# Autodesk Inventor assembly: Caja_Reductora_
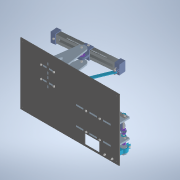
[picture p0: Inventor's stored thumbnail of the model, 180x180]
Saved by Autodesk Inventor 2022 (Build 260153000, 153)
## iProperties
Created: 2022-03-04
Part Number: Caja_Reductora_
Document SubType Name: Assembly
Designer: katha
Author: katha
## Documents named in this file (26)
- C:\Users\katha\OneDrive\Escritorio\Mini_Proyecto_Diseno\Diseno_18012\Modelo_MPD\Caja_Reductora_.iam
- C:\Users\katha\OneDrive\Escritorio\Mini_Proyecto_Diseno\Diseno_18012\Modelo_MPD\Carcasa_CajaR_Lateral1.ipt
- C:\Users\katha\OneDrive\Escritorio\Mini_Proyecto_Diseno\Diseno_18012\Modelo_MPD\Carcasa_Tope.ipt
- C:\Users\katha\OneDrive\Escritorio\Mini_Proyecto_Diseno\Diseno_18012\Modelo_MPD\M4_short.ipt
- C:\Users\katha\OneDrive\Escritorio\Mini_Proyecto_Diseno\Diseno_18012\Modelo_MPD\M4_tuerca.ipt
- C:\Users\katha\OneDrive\Escritorio\Mini_Proyecto_Diseno\Diseno_18012\Modelo_MPD\Rodamiento_Ejes.ipt
- C:\Users\katha\OneDrive\Escritorio\Mini_Proyecto_Diseno\Diseno_18012\Modelo_MPD\Eje_Entrada.ipt
- C:\Users\katha\OneDrive\Escritorio\Mini_Proyecto_Diseno\Diseno_18012\Modelo_MPD\Eje1.ipt
- C:\Users\katha\OneDrive\Escritorio\Mini_Proyecto_Diseno\Diseno_18012\Modelo_MPD\Eje2.ipt
- C:\Users\katha\OneDrive\Escritorio\Mini_Proyecto_Diseno\Diseno_18012\Modelo_MPD\Eje_Salida.ipt
- C:\Users\katha\OneDrive\Escritorio\Mini_Proyecto_Diseno\Diseno_18012\Modelo_MPD\Engranajes_60.ipt
- C:\Users\katha\OneDrive\Escritorio\Mini_Proyecto_Diseno\Diseno_18012\Modelo_MPD\Engranajes_15.ipt
- C:\Users\katha\OneDrive\Escritorio\Mini_Proyecto_Diseno\Diseno_18012\Modelo_MPD\Engranajes_12.ipt
- C:\Users\katha\OneDrive\Escritorio\Mini_Proyecto_Diseno\Diseno_18012\Modelo_MPD\Hombro_Ejes.ipt
- C:\Users\katha\OneDrive\Escritorio\Mini_Proyecto_Diseno\Diseno_18012\Modelo_MPD\pasador.ipt
- C:\Users\katha\OneDrive\Escritorio\Mini_Proyecto_Diseno\Diseno_18012\Modelo_MPD\Base_proyecto.ipt
- C:\Users\katha\OneDrive\Escritorio\Mini_Proyecto_Diseno\Diseno_18012\Modelo_MPD\Base.ipt
- C:\Users\katha\OneDrive\Escritorio\Mini_Proyecto_Diseno\Diseno_18012\Modelo_MPD\Base_Soporte.ipt
- C:\Users\katha\OneDrive\Escritorio\Mini_Proyecto_Diseno\Diseno_18012\Modelo_MPD\Carril.iam
- C:\Users\katha\OneDrive\Escritorio\Mini_Proyecto_Diseno\Diseno_18012\Modelo_MPD\Eslabon_TransPot.ipt
- C:\Users\katha\OneDrive\Escritorio\Mini_Proyecto_Diseno\Diseno_18012\Modelo_MPD\base_motor.ipt
- C:\Users\katha\OneDrive\Escritorio\Mini_Proyecto_Diseno\Diseno_18012\Modelo_MPD\motor.ipt
- C:\Users\katha\OneDrive\Escritorio\Mini_Proyecto_Diseno\Diseno_18012\Modelo_MPD\Acople_TransPot.ipt
- C:\Users\katha\OneDrive\Escritorio\Mini_Proyecto_Diseno\Diseno_18012\Modelo_MPD\Acople_Motor_.ipt
- C:\Users\katha\OneDrive\Escritorio\Mini_Proyecto_Diseno\Diseno_18012\Modelo_MPD\M4_long.ipt
- C:\Users\katha\OneDrive\Escritorio\Mini_Proyecto_Diseno\Diseno_18012\Modelo_MPD\rodamiento_carril.ipt
## Components (99 placed, 25 different names)
1. Carcasa_CajaR_Lateral1:1 — Flush:1, Flush:2, Mate:1, Mate:25, Mate:26, Mate:27, Mate:35, Mate:43, Mate:46, Mate:47, Flush:3, Mate:48, Mate:49, Mate:50, Mate:131, Mate:132, Flush:33
2. Carcasa_CajaR_Lateral1:2 — Flush:1, Flush:2, Mate:1, Mate:28, Mate:29, Mate:30, Mate:44, Mate:45, Mate:51, Mate:52, Mate:53, Mate:54, Flush:4, Mate:141, Mate:142, Mate:143, Mate:144
3. Carcasa_Tope:1 — Mate:25, Mate:26, Mate:27, Mate:33, Mate:34, Mate:36
4. Carcasa_Tope:2 — Mate:28, Mate:29, Mate:30, Mate:31, Mate:32, Mate:37, Mate:38
5. M4_short:1 — Mate:35, Mate:36, Mate:41
6. M4_short:2 — Mate:33, Mate:34, Mate:42
7. M4_short:3 — Mate:37, Mate:38, Mate:39
8. M4_short:4 — Mate:31, Mate:32, Mate:40
9. M4_tuerca:1 — Mate:39, Mate:45
10. M4_tuerca:2 — Mate:40, Mate:44
11. M4_tuerca:3 — Mate:42, Mate:43
12. M4_tuerca:4 — Mate:41, Mate:46
13. Rodamiento_Ejes:1 — Mate:48, Flush:8, Mate:59, Mate:60, Flush:12
14. Rodamiento_Ejes:2 — Mate:49, Flush:9, Mate:63, Mate:64, Flush:13
15. Rodamiento_Ejes:3 — Mate:51, Flush:4, Flush:5, Flush:6, Flush:7, Mate:57, Mate:58
16. Rodamiento_Ejes:4 — Mate:54, Flush:7, Mate:67, Mate:68, Flush:14
17. Rodamiento_Ejes:5 — Mate:53, Flush:6, Mate:65, Mate:66
18. Rodamiento_Ejes:6 — Mate:52, Flush:5, Mate:61, Mate:62
19. Rodamiento_Ejes:7 — Mate:50, Flush:10, Mate:69, Mate:70
20. Rodamiento_Ejes:8 — Mate:47, Flush:3, Flush:8, Flush:9, Flush:10, Mate:55, Mate:56, Flush:11
21. Eje_Entrada:1 — Mate:55, Mate:56, Mate:57, Mate:58, Flush:11, Mate:77, Mate:78, Flush:15, Mate:83, Mate:84, Mate:85, Mate:86, Mate:87, Mate:88, Mate:192, Mate:193, Mate:194
22. Eje1:1 — Mate:59, Mate:60, Mate:61, Mate:62, Flush:12, Mate:73, Mate:74, Mate:79, Mate:80, Flush:17, Mate:89, Mate:90, Mate:91, Mate:92, Mate:93, Mate:94, Mate:95, Mate:96, Mate:97, Mate:98, Mate:99, Mate:100
23. Eje2:1 — Mate:63, Mate:64, Mate:65, Mate:66, Flush:13, Mate:71, Mate:72, Mate:81, Mate:82, Flush:19, Mate:101, Mate:102, Mate:103, Mate:104, Mate:105, Mate:106, Mate:107, Mate:108, Mate:109, Mate:110, Mate:111, Mate:112
24. Eje_Salida:1 — Mate:67, Mate:68, Flush:14, Mate:69, Mate:70, Mate:75, Mate:76, Mate:113, Mate:114, Mate:115, Mate:116, Mate:117, Mate:118, Mate:183, Mate:184, Mate:185
25. Engranajes_60:1 — Mate:71, Mate:72, Flush:18
26. Engranajes_60:2 — Mate:73, Mate:74, Flush:16
27. Engranajes_60:3 — Mate:75, Mate:76, Flush:20
28. Engranajes_15:1 — Mate:77, Mate:78, Flush:15, Flush:16
29. Engranajes_15:2 — Mate:79, Mate:80, Flush:17, Flush:18
30. Engranajes_12:1 — Mate:81, Mate:82, Flush:19, Flush:20
31. Hombro_Ejes:1 — Mate:83, Mate:84, Mate:85, Mate:120, Flush:21
32. Hombro_Ejes:2 — Mate:86, Mate:87, Mate:88, Mate:119, Flush:22
33. Hombro_Ejes:3 — Mate:110, Mate:111, Mate:112, Mate:125, Flush:30
34. Hombro_Ejes:4 — Mate:95, Mate:96, Mate:97, Mate:123, Flush:24
35. Hombro_Ejes:5 — Mate:92, Mate:93, Mate:94, Mate:122, Flush:25
36. Hombro_Ejes:6 — Mate:107, Mate:108, Mate:109, Mate:126, Flush:32
37. Hombro_Ejes:7 — Mate:89, Mate:90, Mate:91, Mate:121, Flush:26
38. Hombro_Ejes:8 — Mate:98, Mate:99, Mate:100, Mate:124, Flush:23
39. Hombro_Ejes:9 — Mate:116, Mate:117, Mate:118, Mate:130, Flush:27
40. Hombro_Ejes:10 — Mate:101, Mate:102, Mate:103, Mate:128, Flush:29
41. Hombro_Ejes:11 — Mate:113, Mate:114, Mate:115, Mate:129, Flush:28
42. Hombro_Ejes:12 — Mate:104, Mate:105, Mate:106, Mate:127, Flush:31
43. pasador:1 — Mate:119, Flush:22
44. pasador:2 — Mate:120, Flush:21
45. pasador:3 — Mate:125, Flush:30
46. pasador:4 — Mate:126, Flush:32
47. pasador:5 — Mate:128, Flush:29
48. pasador:6 — Mate:130, Flush:27
49. pasador:7 — Mate:129, Flush:28
50. pasador:8 — Mate:127, Flush:31
51. pasador:9 — Mate:123, Flush:24
52. pasador:10 — Mate:121, Flush:26
53. pasador:11 — Mate:122, Flush:25
54. pasador:12 — Mate:124, Flush:23
55. Base_proyecto:1 — Mate:131, Mate:132, Flush:33, Mate:133, Mate:134, Mate:135, Mate:136, Mate:137, Mate:138, Mate:139, Mate:140, Mate:149, Mate:150, Mate:151, Mate:152, Flush:34, Flush:35, Mate:153, Mate:154, Flush:36, Mate:155, Mate:156, Mate:157, Mate:158, Mate:159, Mate:160, Mate:161, Mate:162, Mate:179, Mate:180, Mate:181, Mate:218, Mate:219
56. M4_short:5 — Mate:136, Mate:138, Mate:148
57. M4_short:6 — Mate:134, Mate:139, Mate:146
58. M4_short:7 — Mate:133, Mate:137, Mate:147
59. M4_short:8 — Mate:135, Mate:140, Mate:145
60. M4_tuerca:5 — Mate:141, Mate:145
61. M4_tuerca:6 — Mate:144, Mate:147
62. M4_tuerca:7 — Mate:142, Mate:146
63. M4_tuerca:8 — Mate:143, Mate:148
64. Base:1 — Mate:149, Mate:150, Flush:34, Mate:163, Mate:164, Mate:165, Mate:166, Mate:172, Mate:196, Mate:197, Mate:205
65. Base:2 — Mate:151, Mate:152, Flush:35, Mate:171, Mate:203, Mate:204
66. Base_Soporte:1 — Mate:153, Mate:154, Flush:36
67. M4_short:9 — Mate:155, Mate:161, Mate:169
68. M4_short:10 — Mate:156, Mate:159, Mate:170
69. M4_short:11 — Mate:157, Mate:162, Mate:167
70. M4_short:12 — Mate:158, Mate:160, Mate:168
71. M4_tuerca:9 — Mate:163, Mate:169
72. M4_tuerca:10 — Mate:164, Mate:168
73. M4_tuerca:11 — Mate:166, Mate:167
74. M4_tuerca:12 — Mate:165, Mate:170
75. Carril:1 [sub-assembly] — Mate:171, Mate:172, Mate:173, Mate:174, Mate:175, Mate:176, Mate:178, Flush:40
76. Eslabon_TransPot:1 — Mate:173, Mate:174, Mate:186, Mate:187, Mate:188
77. M4_short:13 — Mate:175, Mate:176, Mate:177
78. M4_tuerca:13 — Mate:177, Mate:178
79. base_motor:1 — Mate:179, Mate:180, Mate:181, Flush:37, Mate:182, Mate:208, Mate:209, Mate:211, Mate:212, Mate:213, Mate:214, Mate:215
80. motor:1 — Flush:37, Mate:182
81. Acople_TransPot:1 — Mate:183, Mate:184, Mate:185, Mate:186, Mate:190, Mate:191, Flush:38
82. M4_short:14 — Mate:187, Mate:188, Mate:189
83. M4_tuerca:14 — Mate:189, Mate:190
84. pasador:13 — Mate:191, Flush:38
85. Acople_Motor_:1 — Mate:192, Mate:193, Mate:194, Mate:195, Flush:39
86. pasador:14 — Mate:195, Flush:39
87. M4_long:1 — Mate:196, Mate:197, Mate:198, Mate:199, Mate:200, Mate:201, Mate:202
88. rodamiento_carril:1 — Flush:40, Mate:206, Mate:207
89. M4_tuerca:15 — Mate:198, Mate:206
90. M4_tuerca:16 — Mate:199, Mate:203
91. M4_tuerca:17 — Mate:201, Mate:205
92. M4_tuerca:18 — Mate:200, Mate:204
93. M4_tuerca:19 — Mate:202, Mate:207
94. M4_short:15 — Mate:208, Mate:209, Mate:210
95. M4_tuerca:20 — Mate:210, Mate:211
96. M4_tuerca:21 — Mate:217, Mate:219
97. M4_tuerca:22 — Mate:216, Mate:218
98. M4_short:16 — Mate:212, Mate:215, Mate:217
99. M4_short:17 — Mate:213, Mate:214, Mate:216
## Relationships (236: Mate 196, Flush 40)
- Flush:1: Carcasa_CajaR_Lateral1:1 ↔ Carcasa_CajaR_Lateral1:2
- Flush:2: Carcasa_CajaR_Lateral1:1 ↔ Carcasa_CajaR_Lateral1:2
- Mate:1 (67.8 mm): Carcasa_CajaR_Lateral1:1 ↔ Carcasa_CajaR_Lateral1:2
- Mate:25: Carcasa_CajaR_Lateral1:1 ↔ Carcasa_Tope:1
- Mate:26: Carcasa_CajaR_Lateral1:1 ↔ Carcasa_Tope:1
- Mate:27: Carcasa_CajaR_Lateral1:1 ↔ Carcasa_Tope:1
- Mate:28: Carcasa_CajaR_Lateral1:2 ↔ Carcasa_Tope:2
- Mate:29: Carcasa_CajaR_Lateral1:2 ↔ Carcasa_Tope:2
- Mate:30: Carcasa_CajaR_Lateral1:2 ↔ Carcasa_Tope:2
- Mate:31: Carcasa_Tope:2 ↔ M4_short:4
- Mate:32: Carcasa_Tope:2 ↔ M4_short:4
- Mate:33: Carcasa_Tope:1 ↔ M4_short:2
- Mate:34: Carcasa_Tope:1 ↔ M4_short:2
- Mate:35: Carcasa_CajaR_Lateral1:1 ↔ M4_short:1
- Mate:36: Carcasa_Tope:1 ↔ M4_short:1
- Mate:37: Carcasa_Tope:2 ↔ M4_short:3
- Mate:38: Carcasa_Tope:2 ↔ M4_short:3
- Mate:39: M4_short:3 ↔ M4_tuerca:1
- Mate:40: M4_short:4 ↔ M4_tuerca:2
- Mate:41: M4_short:1 ↔ M4_tuerca:4
- Mate:42: M4_short:2 ↔ M4_tuerca:3
- Mate:43: Carcasa_CajaR_Lateral1:1 ↔ M4_tuerca:3
- Mate:44: Carcasa_CajaR_Lateral1:2 ↔ M4_tuerca:2
- Mate:45: Carcasa_CajaR_Lateral1:2 ↔ M4_tuerca:1
- Mate:46: Carcasa_CajaR_Lateral1:1 ↔ M4_tuerca:4
- Mate:47: Carcasa_CajaR_Lateral1:1 ↔ Rodamiento_Ejes:8
- Flush:3 (0.1 mm): Carcasa_CajaR_Lateral1:1 ↔ Rodamiento_Ejes:8
- Mate:48: Carcasa_CajaR_Lateral1:1 ↔ Rodamiento_Ejes:1
- Mate:49: Carcasa_CajaR_Lateral1:1 ↔ Rodamiento_Ejes:2
- Mate:50: Carcasa_CajaR_Lateral1:1 ↔ Rodamiento_Ejes:7
- Mate:51: Carcasa_CajaR_Lateral1:2 ↔ Rodamiento_Ejes:3
- Mate:52: Carcasa_CajaR_Lateral1:2 ↔ Rodamiento_Ejes:6
- Mate:53: Carcasa_CajaR_Lateral1:2 ↔ Rodamiento_Ejes:5
- Mate:54: Carcasa_CajaR_Lateral1:2 ↔ Rodamiento_Ejes:4
- Flush:4 (-0.1 mm): Carcasa_CajaR_Lateral1:2 ↔ Rodamiento_Ejes:3
- Flush:5: Rodamiento_Ejes:3 ↔ Rodamiento_Ejes:6
- Flush:6: Rodamiento_Ejes:3 ↔ Rodamiento_Ejes:5
- Flush:7: Rodamiento_Ejes:3 ↔ Rodamiento_Ejes:4
- Flush:8: Rodamiento_Ejes:1 ↔ Rodamiento_Ejes:8
- Flush:9: Rodamiento_Ejes:2 ↔ Rodamiento_Ejes:8
- Flush:10: Rodamiento_Ejes:7 ↔ Rodamiento_Ejes:8
- Mate:55 (0.4 mm): Rodamiento_Ejes:8 ↔ Eje_Entrada:1
- Mate:56 (0.4 mm): Rodamiento_Ejes:8 ↔ Eje_Entrada:1
- Mate:57 (0.4 mm): Rodamiento_Ejes:3 ↔ Eje_Entrada:1
- Mate:58 (0.4 mm): Rodamiento_Ejes:3 ↔ Eje_Entrada:1
- Mate:59 (0.4 mm): Rodamiento_Ejes:1 ↔ Eje1:1
- Mate:60 (0.4 mm): Rodamiento_Ejes:1 ↔ Eje1:1
- Mate:61 (0.4 mm): Rodamiento_Ejes:6 ↔ Eje1:1
- Mate:62 (0.4 mm): Rodamiento_Ejes:6 ↔ Eje1:1
- Flush:11: Rodamiento_Ejes:8 ↔ Eje_Entrada:1
- Flush:12: Rodamiento_Ejes:1 ↔ Eje1:1
- Mate:63 (0.4 mm): Rodamiento_Ejes:2 ↔ Eje2:1
- Mate:64 (0.4 mm): Rodamiento_Ejes:2 ↔ Eje2:1
- Mate:65 (0.4 mm): Rodamiento_Ejes:5 ↔ Eje2:1
- Mate:66 (0.4 mm): Rodamiento_Ejes:5 ↔ Eje2:1
- Flush:13: Rodamiento_Ejes:2 ↔ Eje2:1
- Mate:67 (0.4 mm): Rodamiento_Ejes:4 ↔ Eje_Salida:1
- Mate:68 (0.4 mm): Rodamiento_Ejes:4 ↔ Eje_Salida:1
- Flush:14: Rodamiento_Ejes:4 ↔ Eje_Salida:1
- Mate:69 (0.4 mm): Rodamiento_Ejes:7 ↔ Eje_Salida:1
- Mate:70 (0.4 mm): Rodamiento_Ejes:7 ↔ Eje_Salida:1
- Mate:71 (0.5 mm): Eje2:1 ↔ Engranajes_60:1
- Mate:72 (0.5 mm): Eje2:1 ↔ Engranajes_60:1
- Mate:73 (0.5 mm): Eje1:1 ↔ Engranajes_60:2
- Mate:74 (0.5 mm): Eje1:1 ↔ Engranajes_60:2
- Mate:75 (0.5 mm): Eje_Salida:1 ↔ Engranajes_60:3
- Mate:76 (0.5 mm): Eje_Salida:1 ↔ Engranajes_60:3
- Mate:77 (0.5 mm): Eje_Entrada:1 ↔ Engranajes_15:1
- Mate:78 (0.5 mm): Eje_Entrada:1 ↔ Engranajes_15:1
- Mate:79 (0.5 mm): Eje1:1 ↔ Engranajes_15:2
- Mate:80 (0.5 mm): Eje1:1 ↔ Engranajes_15:2
- Mate:81 (0.5 mm): Eje2:1 ↔ Engranajes_12:1
- Mate:82 (0.5 mm): Eje2:1 ↔ Engranajes_12:1
- Flush:15 (55 mm): Eje_Entrada:1 ↔ Engranajes_15:1
- Flush:16: Engranajes_60:2 ↔ Engranajes_15:1
- Flush:17 (20 mm): Eje1:1 ↔ Engranajes_15:2
- Flush:18: Engranajes_60:1 ↔ Engranajes_15:2
- Flush:19 (40 mm): Eje2:1 ↔ Engranajes_12:1
- Flush:20: Engranajes_60:3 ↔ Engranajes_12:1
- Mate:83 (0.45 mm): Eje_Entrada:1 ↔ Hombro_Ejes:1
- Mate:84 (0.45 mm): Eje_Entrada:1 ↔ Hombro_Ejes:1
- Mate:85: Eje_Entrada:1 ↔ Hombro_Ejes:1
- Mate:86 (0.45 mm): Eje_Entrada:1 ↔ Hombro_Ejes:2
- Mate:87 (0.45 mm): Eje_Entrada:1 ↔ Hombro_Ejes:2
- Mate:88: Eje_Entrada:1 ↔ Hombro_Ejes:2
- Mate:89 (0.45 mm): Eje1:1 ↔ Hombro_Ejes:7
- Mate:90 (0.45 mm): Eje1:1 ↔ Hombro_Ejes:7
- Mate:91: Eje1:1 ↔ Hombro_Ejes:7
- Mate:92 (0.45 mm): Eje1:1 ↔ Hombro_Ejes:5
- Mate:93 (0.45 mm): Eje1:1 ↔ Hombro_Ejes:5
- Mate:94: Eje1:1 ↔ Hombro_Ejes:5
- Mate:95 (0.45 mm): Eje1:1 ↔ Hombro_Ejes:4
- Mate:96 (0.45 mm): Eje1:1 ↔ Hombro_Ejes:4
- Mate:97: Eje1:1 ↔ Hombro_Ejes:4
- Mate:98 (0.45 mm): Eje1:1 ↔ Hombro_Ejes:8
- Mate:99 (0.45 mm): Eje1:1 ↔ Hombro_Ejes:8
- Mate:100: Eje1:1 ↔ Hombro_Ejes:8
- Mate:101 (0.45 mm): Eje2:1 ↔ Hombro_Ejes:10
- Mate:102 (0.45 mm): Eje2:1 ↔ Hombro_Ejes:10
- Mate:103: Eje2:1 ↔ Hombro_Ejes:10
- Mate:104 (0.45 mm): Eje2:1 ↔ Hombro_Ejes:12
- Mate:105 (0.45 mm): Eje2:1 ↔ Hombro_Ejes:12
- Mate:106: Eje2:1 ↔ Hombro_Ejes:12
- Mate:107 (0.45 mm): Eje2:1 ↔ Hombro_Ejes:6
- Mate:108 (0.45 mm): Eje2:1 ↔ Hombro_Ejes:6
- Mate:109: Eje2:1 ↔ Hombro_Ejes:6
- Mate:110 (0.45 mm): Eje2:1 ↔ Hombro_Ejes:3
- Mate:111 (0.45 mm): Eje2:1 ↔ Hombro_Ejes:3
- Mate:112: Eje2:1 ↔ Hombro_Ejes:3
- Mate:113 (0.45 mm): Eje_Salida:1 ↔ Hombro_Ejes:11
- Mate:114 (0.45 mm): Eje_Salida:1 ↔ Hombro_Ejes:11
- Mate:115: Eje_Salida:1 ↔ Hombro_Ejes:11
- Mate:116 (0.45 mm): Eje_Salida:1 ↔ Hombro_Ejes:9
- Mate:117 (0.45 mm): Eje_Salida:1 ↔ Hombro_Ejes:9
- Mate:118: Eje_Salida:1 ↔ Hombro_Ejes:9
- Mate:119: Hombro_Ejes:2 ↔ pasador:1
- Mate:120: Hombro_Ejes:1 ↔ pasador:2
- Mate:121: Hombro_Ejes:7 ↔ pasador:10
- Mate:122: Hombro_Ejes:5 ↔ pasador:11
- Mate:123: Hombro_Ejes:4 ↔ pasador:9
- Mate:124: Hombro_Ejes:8 ↔ pasador:12
- Mate:125: Hombro_Ejes:3 ↔ pasador:3
- Mate:126: Hombro_Ejes:6 ↔ pasador:4
- Mate:127: Hombro_Ejes:12 ↔ pasador:8
- Mate:128: Hombro_Ejes:10 ↔ pasador:5
- Mate:129: Hombro_Ejes:11 ↔ pasador:7
- Mate:130: Hombro_Ejes:9 ↔ pasador:6
- Flush:21: Hombro_Ejes:1 ↔ pasador:2
- Flush:22: Hombro_Ejes:2 ↔ pasador:1
- Flush:23: Hombro_Ejes:8 ↔ pasador:12
- Flush:24: Hombro_Ejes:4 ↔ pasador:9
- Flush:25: Hombro_Ejes:5 ↔ pasador:11
- Flush:26: Hombro_Ejes:7 ↔ pasador:10
- Flush:27: Hombro_Ejes:9 ↔ pasador:6
- Flush:28: Hombro_Ejes:11 ↔ pasador:7
- Flush:29: Hombro_Ejes:10 ↔ pasador:5
- Flush:30: Hombro_Ejes:3 ↔ pasador:3
- Flush:31: Hombro_Ejes:12 ↔ pasador:8
- Flush:32: Hombro_Ejes:6 ↔ pasador:4
- Mate:131: Carcasa_CajaR_Lateral1:1 ↔ Base_proyecto:1
- Mate:132: Carcasa_CajaR_Lateral1:1 ↔ Base_proyecto:1
- Flush:33: Carcasa_CajaR_Lateral1:1 ↔ Base_proyecto:1
- Mate:133: Base_proyecto:1 ↔ M4_short:7
- Mate:134: Base_proyecto:1 ↔ M4_short:6
- Mate:135: Base_proyecto:1 ↔ M4_short:8
- Mate:136: Base_proyecto:1 ↔ M4_short:5
- Mate:137: Base_proyecto:1 ↔ M4_short:7
- Mate:138: Base_proyecto:1 ↔ M4_short:5
- Mate:139: Base_proyecto:1 ↔ M4_short:6
- Mate:140: Base_proyecto:1 ↔ M4_short:8
- Mate:141: Carcasa_CajaR_Lateral1:2 ↔ M4_tuerca:5
- Mate:142: Carcasa_CajaR_Lateral1:2 ↔ M4_tuerca:7
- Mate:143: Carcasa_CajaR_Lateral1:2 ↔ M4_tuerca:8
- Mate:144: Carcasa_CajaR_Lateral1:2 ↔ M4_tuerca:6
- Mate:145: M4_short:8 ↔ M4_tuerca:5
- Mate:146: M4_short:6 ↔ M4_tuerca:7
- Mate:147: M4_short:7 ↔ M4_tuerca:6
- Mate:148: M4_short:5 ↔ M4_tuerca:8
- Mate:149: Base_proyecto:1 ↔ Base:1
- Mate:150: Base_proyecto:1 ↔ Base:1
- Mate:151: Base_proyecto:1 ↔ Base:2
- Mate:152: Base_proyecto:1 ↔ Base:2
- Flush:34: Base_proyecto:1 ↔ Base:1
- Flush:35: Base_proyecto:1 ↔ Base:2
- Mate:153: Base_proyecto:1 ↔ Base_Soporte:1
- Mate:154: Base_proyecto:1 ↔ Base_Soporte:1
- Flush:36: Base_proyecto:1 ↔ Base_Soporte:1
- Mate:155: Base_proyecto:1 ↔ M4_short:9
- Mate:156: Base_proyecto:1 ↔ M4_short:10
- Mate:157: Base_proyecto:1 ↔ M4_short:11
- Mate:158: Base_proyecto:1 ↔ M4_short:12
- Mate:159: Base_proyecto:1 ↔ M4_short:10
- Mate:160: Base_proyecto:1 ↔ M4_short:12
- Mate:161: Base_proyecto:1 ↔ M4_short:9
- Mate:162: Base_proyecto:1 ↔ M4_short:11
- Mate:163: Base:1 ↔ M4_tuerca:9
- Mate:164: Base:1 ↔ M4_tuerca:10
- Mate:165: Base:1 ↔ M4_tuerca:12
- Mate:166: Base:1 ↔ M4_tuerca:11
- Mate:167: M4_short:11 ↔ M4_tuerca:11
- Mate:168: M4_short:12 ↔ M4_tuerca:10
- Mate:169: M4_short:9 ↔ M4_tuerca:9
- Mate:170: M4_short:10 ↔ M4_tuerca:12
- Mate:171: Base:2 ↔ Carril:1
- Mate:172 (18.25 mm): Base:1 ↔ Carril:1
- Mate:173: Carril:1 ↔ Eslabon_TransPot:1
- Mate:174 (0.3 mm): Carril:1 ↔ Eslabon_TransPot:1
- Mate:175: Carril:1 ↔ M4_short:13
- Mate:176: Carril:1 ↔ M4_short:13
- Mate:177: M4_short:13 ↔ M4_tuerca:13
- Mate:178: Carril:1 ↔ M4_tuerca:13
- Mate:179: Base_proyecto:1 ↔ base_motor:1
- Mate:180: Base_proyecto:1 ↔ base_motor:1
- Mate:181: Base_proyecto:1 ↔ base_motor:1
- Flush:37 (-8 mm): base_motor:1 ↔ motor:1
- Mate:182: base_motor:1 ↔ motor:1
- Mate:183 (0.4 mm): Eje_Salida:1 ↔ Acople_TransPot:1
- Mate:184 (0.4 mm): Eje_Salida:1 ↔ Acople_TransPot:1
- Mate:185: Eje_Salida:1 ↔ Acople_TransPot:1
- Mate:186: Eslabon_TransPot:1 ↔ Acople_TransPot:1
- Mate:187: Eslabon_TransPot:1 ↔ M4_short:14
- Mate:188: Eslabon_TransPot:1 ↔ M4_short:14
- Mate:189: M4_short:14 ↔ M4_tuerca:14
- Mate:190: Acople_TransPot:1 ↔ M4_tuerca:14
- Mate:191: Acople_TransPot:1 ↔ pasador:13
- Flush:38: Acople_TransPot:1 ↔ pasador:13
- Mate:192 (0.4 mm): Eje_Entrada:1 ↔ Acople_Motor_:1
- Mate:193 (0.4 mm): Eje_Entrada:1 ↔ Acople_Motor_:1
- Mate:194: Eje_Entrada:1 ↔ Acople_Motor_:1
- Mate:195: Acople_Motor_:1 ↔ pasador:14
- Flush:39: Acople_Motor_:1 ↔ pasador:14
- Mate:196: Base:1 ↔ M4_long:1
- Mate:197: Base:1 ↔ M4_long:1
- Flush:40: Carril:1 ↔ rodamiento_carril:1
- Mate:198: M4_long:1 ↔ M4_tuerca:15
- Mate:199: M4_long:1 ↔ M4_tuerca:16
- Mate:200: M4_long:1 ↔ M4_tuerca:18
- Mate:201: M4_long:1 ↔ M4_tuerca:17
- Mate:202: M4_long:1 ↔ M4_tuerca:19
- Mate:203: Base:2 ↔ M4_tuerca:16
- Mate:204: Base:2 ↔ M4_tuerca:18
- Mate:205: Base:1 ↔ M4_tuerca:17
- Mate:206: rodamiento_carril:1 ↔ M4_tuerca:15
- Mate:207: rodamiento_carril:1 ↔ M4_tuerca:19
- Mate:208: base_motor:1 ↔ M4_short:15
- Mate:209: base_motor:1 ↔ M4_short:15
- Mate:210: M4_short:15 ↔ M4_tuerca:20
- Mate:211: base_motor:1 ↔ M4_tuerca:20
- Mate:212: base_motor:1 ↔ M4_short:16
- Mate:213: base_motor:1 ↔ M4_short:17
- Mate:214: base_motor:1 ↔ M4_short:17
- Mate:215: base_motor:1 ↔ M4_short:16
- Mate:216: M4_tuerca:22 ↔ M4_short:17
- Mate:217: M4_tuerca:21 ↔ M4_short:16
- Mate:218: Base_proyecto:1 ↔ M4_tuerca:22
- Mate:219: Base_proyecto:1 ↔ M4_tuerca:21
